# Autodesk Inventor assembly: wszystkie scianki
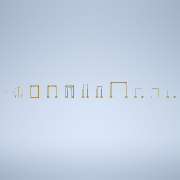
[picture p0: Inventor's stored thumbnail of the model, 180x180]
Saved by Autodesk Inventor 2021 (Build 250183000, 183)
## iProperties
Created: 2024-04-21
Part Number: wszystkie scianki
Document SubType Name: Assembly
Designer: Michal
Author: Michal
## Documents named in this file (12)
- C:\Users\Michal\Documents\GitHub\PNW_PhotoBoothFrame_3D\wszystkie scianki.iam
- C:\Users\Michal\Documents\GitHub\PNW_PhotoBoothFrame_3D\prostkatna waska wysoka kwadraty.iam
- C:\Users\Michal\Documents\GitHub\PNW_PhotoBoothFrame_3D\prostkatna waska wysoka lacznik.iam
- C:\Users\Michal\Documents\GitHub\PNW_PhotoBoothFrame_3D\prostkatna waska niska kwadraty.iam
- C:\Users\Michal\Documents\GitHub\PNW_PhotoBoothFrame_3D\prostkatna szeroka wysoka kwadraty.iam
- C:\Users\Michal\Documents\GitHub\PNW_PhotoBoothFrame_3D\zaokraglona waska wysoka kwadraty.iam
- C:\Users\Michal\Documents\GitHub\PNW_PhotoBoothFrame_3D\pol zaokraglona waska wysoka kwadraty.iam
- C:\Users\Michal\Documents\GitHub\PNW_PhotoBoothFrame_3D\brama kwadraty.iam
- C:\Users\Michal\Documents\GitHub\PNW_PhotoBoothFrame_3D\prostkatna waska niska kwadraty v2.iam
- C:\Users\Michal\Documents\GitHub\PNW_PhotoBoothFrame_3D\prostkatna waska wysoka lacznik v2.iam
- C:\Users\Michal\Documents\GitHub\PNW_PhotoBoothFrame_3D\okragla duza.iam
- C:\Users\Michal\Documents\GitHub\PNW_PhotoBoothFrame_3D\okragla mala napis.iam
## Components (11 placed, 11 different names)
1. prostkatna waska wysoka kwadraty:1 [sub-assembly] — Flush:1, Flush:2, Mate:1, Flush:5, Flush:6, Mate:3
2. prostkatna waska wysoka lacznik:1 [sub-assembly] — Flush:1, Flush:2, Mate:1, Flush:3, Flush:4, Mate:2
3. prostkatna waska niska kwadraty:1 [sub-assembly] — Flush:3, Flush:4, Mate:2
4. prostkatna szeroka wysoka kwadraty:1 [sub-assembly] — Flush:5, Flush:6, Mate:3, Flush:7, Flush:8, Mate:4
5. zaokraglona waska wysoka kwadraty:1 [sub-assembly] — Flush:7, Flush:8, Mate:4, Flush:9, Flush:10, Mate:5
6. pol zaokraglona waska wysoka kwadraty:1 [sub-assembly] — Flush:9, Flush:10, Mate:5, Flush:11, Flush:12, Mate:6
7. brama kwadraty:1 [sub-assembly] — Flush:11, Flush:12, Mate:6, Flush:13, Flush:14, Mate:7
8. prostkatna waska niska kwadraty v2:1 [sub-assembly] — Flush:13, Flush:14, Mate:7, Flush:15, Flush:16, Mate:8
9. prostkatna waska wysoka lacznik v2:1 [sub-assembly] — Flush:15, Flush:16, Mate:8, Flush:17, Flush:18, Mate:9
10. okragla duza:1 [sub-assembly] — Flush:17, Flush:18, Mate:9, Flush:19, Mate:10
11. okragla mala napis:1 [sub-assembly] — Flush:19, Mate:10
## Relationships (29: Flush 19, Mate 10)
- Flush:1: prostkatna waska wysoka kwadraty:1 ↔ prostkatna waska wysoka lacznik:1
- Flush:2: prostkatna waska wysoka kwadraty:1 ↔ prostkatna waska wysoka lacznik:1
- Mate:1 (2000 mm): prostkatna waska wysoka kwadraty:1 ↔ prostkatna waska wysoka lacznik:1
- Flush:3: prostkatna waska wysoka lacznik:1 ↔ prostkatna waska niska kwadraty:1
- Flush:4: prostkatna waska wysoka lacznik:1 ↔ prostkatna waska niska kwadraty:1
- Mate:2 (2000 mm): prostkatna waska wysoka lacznik:1 ↔ prostkatna waska niska kwadraty:1
- Flush:5: prostkatna waska wysoka kwadraty:1 ↔ prostkatna szeroka wysoka kwadraty:1
- Flush:6: prostkatna waska wysoka kwadraty:1 ↔ prostkatna szeroka wysoka kwadraty:1
- Mate:3 (2000 mm): prostkatna waska wysoka kwadraty:1 ↔ prostkatna szeroka wysoka kwadraty:1
- Flush:7: prostkatna szeroka wysoka kwadraty:1 ↔ zaokraglona waska wysoka kwadraty:1
- Flush:8: prostkatna szeroka wysoka kwadraty:1 ↔ zaokraglona waska wysoka kwadraty:1
- Mate:4 (2000 mm): prostkatna szeroka wysoka kwadraty:1 ↔ zaokraglona waska wysoka kwadraty:1
- Flush:9: zaokraglona waska wysoka kwadraty:1 ↔ pol zaokraglona waska wysoka kwadraty:1
- Flush:10: zaokraglona waska wysoka kwadraty:1 ↔ pol zaokraglona waska wysoka kwadraty:1
- Mate:5 (2000 mm): zaokraglona waska wysoka kwadraty:1 ↔ pol zaokraglona waska wysoka kwadraty:1
- Flush:11: pol zaokraglona waska wysoka kwadraty:1 ↔ brama kwadraty:1
- Flush:12: pol zaokraglona waska wysoka kwadraty:1 ↔ brama kwadraty:1
- Mate:6 (2000 mm): pol zaokraglona waska wysoka kwadraty:1 ↔ brama kwadraty:1
- Flush:13: brama kwadraty:1 ↔ prostkatna waska niska kwadraty v2:1
- Flush:14: brama kwadraty:1 ↔ prostkatna waska niska kwadraty v2:1
- Mate:7 (2000 mm): brama kwadraty:1 ↔ prostkatna waska niska kwadraty v2:1
- Flush:15: prostkatna waska niska kwadraty v2:1 ↔ prostkatna waska wysoka lacznik v2:1
- Flush:16: prostkatna waska niska kwadraty v2:1 ↔ prostkatna waska wysoka lacznik v2:1
- Mate:8 (2000 mm): prostkatna waska niska kwadraty v2:1 ↔ prostkatna waska wysoka lacznik v2:1
- Flush:17: prostkatna waska wysoka lacznik v2:1 ↔ okragla duza:1
- Flush:18: prostkatna waska wysoka lacznik v2:1 ↔ okragla duza:1
- Mate:9 (2000 mm): prostkatna waska wysoka lacznik v2:1 ↔ okragla duza:1
- Flush:19: okragla duza:1 ↔ okragla mala napis:1
- Mate:10 (2000 mm): okragla duza:1 ↔ okragla mala napis:1
